# Autodesk Inventor assembly: Wrist
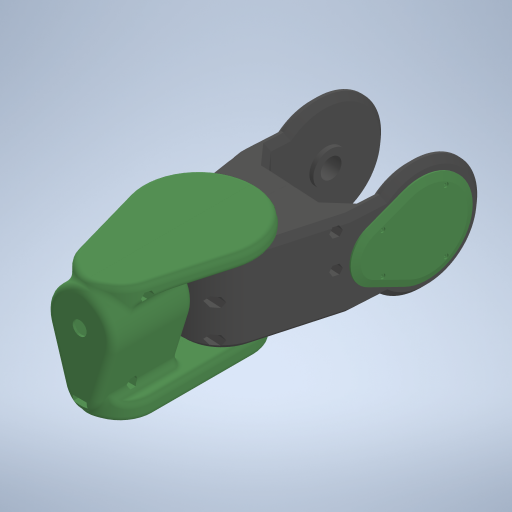
[picture p0: Inventor's stored thumbnail of the model, 512x512]
Saved by Autodesk Inventor 2023 (Build 270158000, 158)
## iProperties
Created: 2024-07-25
Part Number: Wrist
Document SubType Name: Assembly
Designer: Swoby
Author: Swoby
## Documents named in this file (6)
- C:\Users\Swoby\OneDrive\Plocha\DUM-E\V0.3\NewWirst\Wrist.iam
- C:\Users\Swoby\OneDrive\Plocha\DUM-E\V0.3\NewWirst\Wirst_1L.ipt
- C:\Users\Swoby\OneDrive\Plocha\DUM-E\V0.3\NewWirst\Wirst_1R.ipt
- C:\Users\Swoby\OneDrive\Plocha\DUM-E\V0.3\NewWirst\Wirst_2R.ipt
- C:\Users\Swoby\OneDrive\Plocha\DUM-E\V0.3\NewWirst\Wirst_2R_cover.ipt
- C:\Users\Swoby\OneDrive\Plocha\DUM-E\V0.3\NewWirst\Wirst_2L.ipt
## Components (6 placed, 5 different names)
1. Wirst_1L:1 — Mate:1, Mate:2, Mate:4
2. Wirst_1R:1 — Mate:1, Mate:2, Mate:3, Mate:4, Mate:5
3. Wirst_2R:1 — Mate:3, Mate:5, Mate:6, Mate:8, Mate:9, Mate:10, Mate:11, Mate:12
4. Wirst_2R_cover:1 — Mate:6, Mate:11, Mate:12
5. Wirst_2L:1 — Mate:8, Mate:9, Mate:10, Mate:13, Mate:14, Mate:15
6. Wirst_2R_cover:2 — Mate:13, Mate:14, Mate:15
## Relationships (14: Mate 14)
- Mate:1: Wirst_1L:1 ↔ Wirst_1R:1
- Mate:2: Wirst_1L:1 ↔ Wirst_1R:1
- Mate:3: Wirst_1R:1 ↔ Wirst_2R:1
- Mate:4: Wirst_1L:1 ↔ Wirst_1R:1
- Mate:5 (0.5 mm): Wirst_1R:1 ↔ Wirst_2R:1
- Mate:6: Wirst_2R:1 ↔ Wirst_2R_cover:1
- Mate:8: Wirst_2R:1 ↔ Wirst_2L:1
- Mate:9: Wirst_2R:1 ↔ Wirst_2L:1
- Mate:10: Wirst_2R:1 ↔ Wirst_2L:1
- Mate:11: Wirst_2R:1 ↔ Wirst_2R_cover:1
- Mate:12: Wirst_2R:1 ↔ Wirst_2R_cover:1
- Mate:13: Wirst_2L:1 ↔ Wirst_2R_cover:2
- Mate:14: Wirst_2L:1 ↔ Wirst_2R_cover:2
- Mate:15: Wirst_2L:1 ↔ Wirst_2R_cover:2
